# Autodesk Inventor assembly: Assy
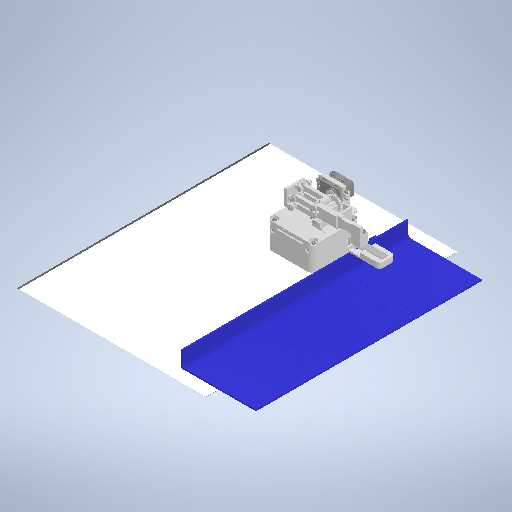
[picture p0: Inventor's stored thumbnail of the model, 512x512]
Saved by Autodesk Inventor 2025 (Build 290162000, 162)
## iProperties
Created: 2026-02-16
Part Number: Assy
Document SubType Name: Assembly
Designer: sooo1
Author: sooo1
## Documents named in this file (3)
- C:\Users\sooo1\Downloads\final-20260216T060151Z-1-001\final\Assy.iam
- C:\Users\sooo1\Downloads\final-20260216T060151Z-1-001\final\MOBITOUCH.iam
- C:\Users\sooo1\Downloads\final-20260216T060151Z-1-001\final\field\field.iam
## Components (2 placed, 2 different names)
1. MOBITOUCH:1 [sub-assembly] — フラッシュ:4, 角度:1, メイト:1
2. field:1 [sub-assembly] — フラッシュ:1, フラッシュ:2, フラッシュ:3, フラッシュ:4, メイト:1
## Relationships (6: Flush 4, Angle 1, Mate 1)
- フラッシュ:1 [Flush]: field:1
- フラッシュ:2 [Flush]: field:1
- フラッシュ:3 [Flush]: field:1
- フラッシュ:4 [Flush]: MOBITOUCH:1 ↔ field:1
- 角度:1 [Angle] (180 deg): MOBITOUCH:1
- メイト:1 [Mate] (20 mm): MOBITOUCH:1 ↔ field:1
